# Autodesk Inventor assembly: FEM-Träger-Baugruppe4
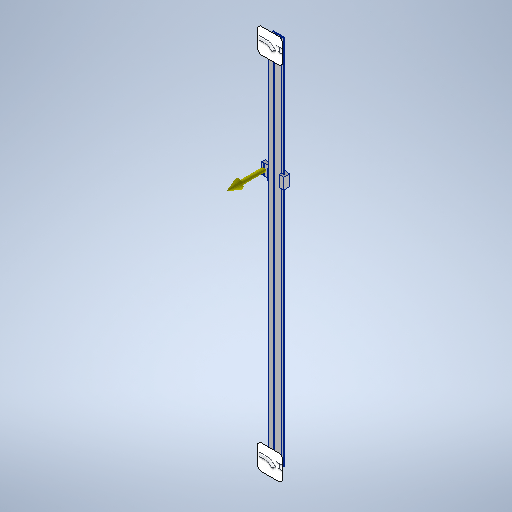
[picture p0: Inventor's stored thumbnail of the model, 512x512]
Saved by Autodesk Inventor 2025 (Build 290162010, 162A)
## iProperties
Created: 2025-02-05
Part Number: FEM-Träger-Baugruppe4
Document SubType Name: Assembly
Designer: Admin
Mass: 496.826 g
Surface Area: 1700.01 cm^2
Volume: 184.01 cm^3
Density: 2.7 g/cm^3
Author: Admin
## Documents named in this file (17)
- C:\Users\Admin\GIT\HDVKBM\CAD\Krandemonstrator\FEM-Träger-Baugruppe7.iam
- C:\Users\Admin\GIT\HDVKBM\CAD\Krandemonstrator\TrägerUI.ipt
- C:\Users\Admin\GIT\HDVKBM\CAD\Krandemonstrator\KatzeFEM.ipt
- C:\Users\Admin\GIT\HDVKBM\CAD\Krandemonstrator\FEM-Träger-Baugruppe7\AIP\FEA\eywnjn6hs.fins
- C:\Users\Admin\GIT\HDVKBM\CAD\Krandemonstrator\FEM-Träger-Baugruppe7\AIP\FEA\eywnjn6hs.fsat
- C:\Users\Admin\GIT\HDVKBM\CAD\Krandemonstrator\FEM-Träger-Baugruppe7\AIP\FEA\eywnjn6io.ftes
- C:\Users\Admin\GIT\HDVKBM\CAD\Krandemonstrator\FEM-Träger-Baugruppe7\AIP\FEA\eywnjn6io.fwiz
- C:\Users\Admin\GIT\HDVKBM\CAD\Krandemonstrator\FEM-Träger-Baugruppe7\AIP\FEA\eywnjn6m8.fmsh
- C:\Users\Admin\GIT\HDVKBM\CAD\Krandemonstrator\FEM-Träger-Baugruppe7\AIP\FEA\eywug1khs.fmsh
- C:\Users\Admin\GIT\HDVKBM\CAD\Krandemonstrator\FEM-Träger-Baugruppe7\AIP\FEA\eywug1kht.fres
- C:\Users\Admin\GIT\HDVKBM\CAD\Krandemonstrator\FEM-Träger-Baugruppe7\AIP\FEA\eywug1kkg.fmsh
- C:\Users\Admin\GIT\HDVKBM\CAD\Krandemonstrator\FEM-Träger-Baugruppe7\AIP\FEA\eywug1kkh.fres
- C:\Users\Admin\GIT\HDVKBM\CAD\Krandemonstrator\FEM-Träger-Baugruppe7\AIP\FEA\eywuzuqqo.fmsh
- C:\Users\Admin\GIT\HDVKBM\CAD\Krandemonstrator\FEM-Träger-Baugruppe7\AIP\FEA\eywuzuqsg.fmsh
- C:\Users\Admin\GIT\HDVKBM\CAD\Krandemonstrator\FEM-Träger-Baugruppe7\AIP\FEA\eywuzuqu8.fmsh
- C:\Users\Admin\GIT\HDVKBM\CAD\Krandemonstrator\FEM-Träger-Baugruppe7\AIP\FEA\eywuzuqww.fmsh
- C:\Users\Admin\GIT\HDVKBM\CAD\Krandemonstrator\FEM-Träger-Baugruppe7\AIP\FEA\eywuzuqwx.fres
## Components (2 placed, 2 different names)
1. TrägerUI:1 — Verschiebbar:1
2. KatzeFEM:1 — Verschiebbar:1
## Relationships (1: TranslationJoint 1)
- Verschiebbar:1 [TranslationJoint] (1 mm): TrägerUI:1 ↔ KatzeFEM:1
## Named parameters: sa_0 = 25000, sa_1 = 25000, sa_2 = 25000, sa_3 = 25000, sa_4 = 25000, sa_5 = 25000, sa_6 = 25000, sa_7 = 50000
note: some values were not read from the file. Shown as the stored number, unit unknown: "sa_0", "sa_1", "sa_2", "sa_3", "sa_4", "sa_5", "sa_6", "sa_7".
